# Autodesk Inventor assembly: TI-83x
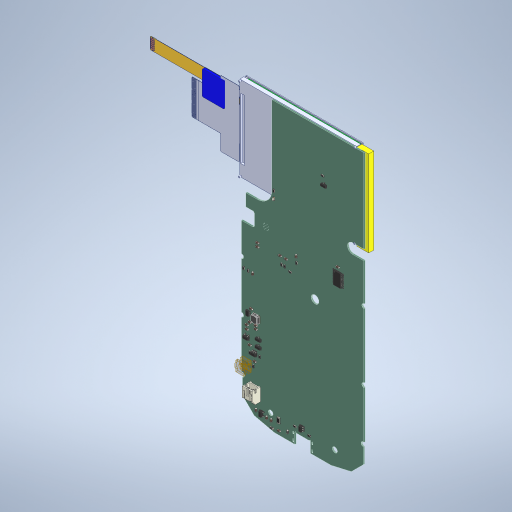
[picture p0: Inventor's stored thumbnail of the model, 512x512]
Saved by Autodesk Inventor 2023 (Build 270158000, 158)
## iProperties
Created: 2023-03-09
Part Number: TI-83x
Document SubType Name: Assembly
Designer: Peter
Title: TI-83x
Author: Peter
## Documents named in this file (4)
- D:\Documents\KiCad\6.0\projects\TI-83x\CAD\TI-83x.iam
- D:\Documents\KiCad\6.0\projects\TI-83x\CAD\TI-83x.ipt
- D:\Documents\KiCad\6.0\projects\TI-83x\CAD\NHD-2.8-240320AF-CSXP-F-CTP.ipt
- D:\Documents\KiCad\6.0\projects\TI-83x\CAD\LeftScreenSpacer.ipt
## Components (3 placed, 3 different names)
1. TI-83x_PCB:1 — Mate:1, Flush:1, Mate:2, Flush:2
2. NHD-2.8-240320AF-CSXP-F-CTP:1 — Mate:1, Flush:1, Mate:3
3. LeftScreenSpacer:1 — Mate:2, Flush:2, Mate:3
## Relationships (5: Mate 3, Flush 2)
- Mate:1: TI-83x_PCB:1 ↔ NHD-2.8-240320AF-CSXP-F-CTP:1
- Flush:1 (5.08 mm): TI-83x_PCB:1 ↔ NHD-2.8-240320AF-CSXP-F-CTP:1
- Mate:2: TI-83x_PCB:1 ↔ LeftScreenSpacer:1
- Flush:2: TI-83x_PCB:1 ↔ LeftScreenSpacer:1
- Mate:3: NHD-2.8-240320AF-CSXP-F-CTP:1 ↔ LeftScreenSpacer:1
